# Autodesk Inventor assembly: 2.75 Omni AS, No Insert_MIR
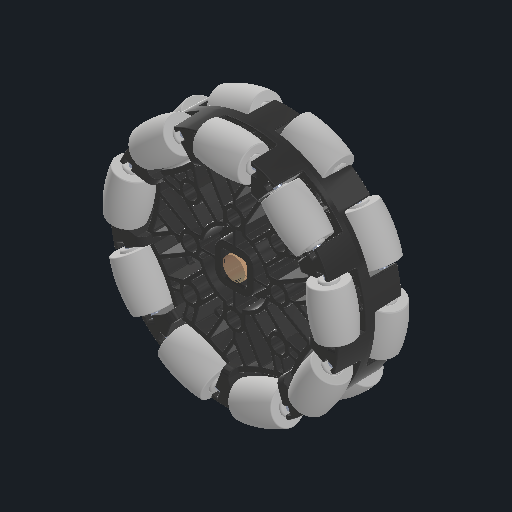
[picture p0: Inventor's stored thumbnail of the model, 512x512]
Saved by Autodesk Inventor 2024 (Build 280153000, 153)
## iProperties
Created: 2022-08-02
Part Number: 2.75 Omni AS, No Insert_MIR
Document SubType Name: Assembly
Designer: avere
Author: ylu12
## Documents named in this file (2)
- C:\Users\avere\Documents\rbp_cad\zoomba_v0.1\chassis\mirrored_parts\2.75 Omni AS, No Insert_MIR.iam
- C:\Users\avere\Documents\rbp_cad\zoomba_v0.1\chassis\mirrored_parts\2.75 Omni Antistatic_MIR.ipt
## Components (1 placed, 1 different names)
1. 2.75 Omni Antistatic_MIR:1 — Mate:8, Mate:7, Flush:4
## Relationships (3: Mate 2, Flush 1)
- Mate:8: 2.75 Omni Antistatic_MIR:1
- Mate:7: 2.75 Omni Antistatic_MIR:1
- Flush:4: 2.75 Omni Antistatic_MIR:1
